# Autodesk Inventor assembly: ND Motor Right 1764
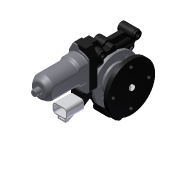
[picture p0: Inventor's stored thumbnail of the model, 180x180]
Saved by Autodesk Inventor 2011 (Build 150239000, 239)
## iProperties
Shininess: 64.0
Length Units: 11272
Angle Units: 11279
Time Units: 11290
Mass Units: 11286
Length Display Precision: 3
Angle Display Precision: 2
Compacted: True
Part Number: ND Motor Right 1764
Document SubType Name: Assembly
Created: 2006-01-29
Designer: Ed Sparks
Density: 0.0
Volumn: 0.0
Area: 0.0
PropertySet Name: Model Information
Control State: 0
Master: False
Checked Out: False
Author: Ed Sparks
## Documents named in this file (3)
- R:\2010-2011\CMO\Web Site\CADalog\Motors\ND Motor Right 1764.iam
- R:\CAD Archives\Motors\ND Motor Right 1764\ND Motor Right 1764.ipt
- R:\CAD Archives\Motors\ND Motor Right 1764\Window Motor Coupler 2 1764.ipt
## Components (2 placed, 2 different names)
1. ND Motor Right 1764:1 — Angle:1, Mate:2, Mate:3, Mate:4
2. Window Motor Coupler 2 1764:1 — Angle:1, Mate:2, Mate:3, Mate:4
## Relationships (4: Mate 3, Angle 1)
- Angle:1 (60 deg): ND Motor Right 1764:1 ↔ Window Motor Coupler 2 1764:1
- Mate:2: ND Motor Right 1764:1 ↔ Window Motor Coupler 2 1764:1
- Mate:3: ND Motor Right 1764:1 ↔ Window Motor Coupler 2 1764:1
- Mate:4: ND Motor Right 1764:1 ↔ Window Motor Coupler 2 1764:1
